# Autodesk Inventor assembly: Lidar Sensor Case Assembly v2
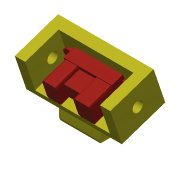
[picture p0: Inventor's stored thumbnail of the model, 180x180]
Saved by Autodesk Inventor 2018.3 (Build 223284000, 284)
## iProperties
Created: 2019-02-08
Part Number: Lidar Sensor Case Assembly v2
Document SubType Name: Assembly
Designer: aye06091
Mass: 28.242 g
Surface Area: 134.46 cm^2
Volume: 28.242 cm^3
Density: 1 g/cm^3
Author: aye06091
## Documents named in this file (3)
- Y:\DeSimony-R\Senior R&D\4 R&D Shared Folder\VisiStick\VisiStick (Inventor)\Physical Parts\Lidar Sensor Case Assembly v2.iam
- Y:\DeSimony-R\Senior R&D\4 R&D Shared Folder\VisiStick\VisiStick (Inventor)\Electronics\Sharp 2Y0A02.ipt
- Y:\DeSimony-R\Senior R&D\4 R&D Shared Folder\VisiStick\VisiStick (Inventor)\Physical Parts\Lidar Sensor Case v2.ipt
## Components (2 placed, 2 different names)
1. Sharp 2Y0A02:1 — Mate:1, Mate:2, Mate:3
2. Lidar Sensor Case v2:1 — Mate:1, Mate:2, Mate:3
## Relationships (3: Mate 3)
- Mate:1 (1.27 mm): Sharp 2Y0A02:1 ↔ Lidar Sensor Case v2:1
- Mate:2: Sharp 2Y0A02:1 ↔ Lidar Sensor Case v2:1
- Mate:3: Sharp 2Y0A02:1 ↔ Lidar Sensor Case v2:1
